# Autodesk Inventor assembly: MQ135
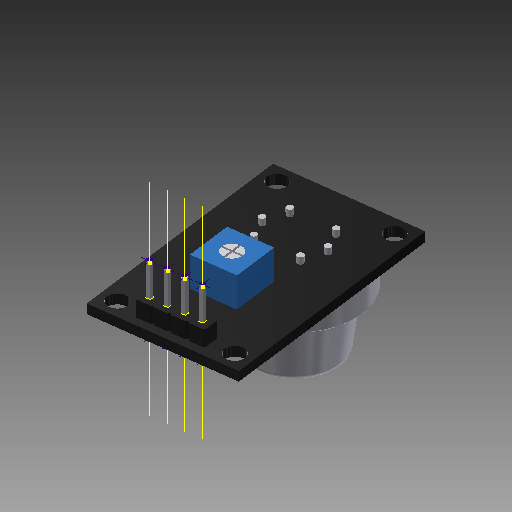
[picture p0: Inventor's stored thumbnail of the model, 512x512]
Saved by Autodesk Inventor 2019 (Build 230136000, 136)
## iProperties
Created: 2019-06-05
Part Number: MQ135
Material: Generisch
Document SubType Name: Assembly
Designer: manue
Author: manue
## Documents named in this file (5)
- E:\Benutzer\manue\Nextcloud\Unterlagen\Studium\OTH AMBERG\Industrie 4.0\Semester 4\Projektmanagement & agile Projektmethoden\Projekt Sensornetzwerk\Sensorknoten\Modell\MQ135\MQ135.iam
- E:\Benutzer\manue\Nextcloud\Unterlagen\Studium\OTH AMBERG\Industrie 4.0\Semester 4\Projektmanagement & agile Projektmethoden\Projekt Sensornetzwerk\Sensorknoten\Modell\MQ135\User Library-MQ135.ipt
- E:\Benutzer\manue\Nextcloud\Unterlagen\Studium\OTH AMBERG\Industrie 4.0\Semester 4\Projektmanagement & agile Projektmethoden\Projekt Sensornetzwerk\Sensorknoten\Modell\MQ135\Platine.ipt
- E:\Benutzer\manue\Nextcloud\Unterlagen\Studium\OTH AMBERG\Industrie 4.0\Semester 4\Projektmanagement & agile Projektmethoden\Projekt Sensornetzwerk\Sensorknoten\Modell\MQ135\Kontaktpins_Gerade.iam
- E:\Benutzer\manue\Nextcloud\Unterlagen\Studium\OTH AMBERG\Industrie 4.0\Semester 4\Projektmanagement & agile Projektmethoden\Projekt Sensornetzwerk\Sensorknoten\Modell\MQ135\Poti.ipt
## Components (7 placed, 4 different names)
1. User Library-MQ135:1 — Passend:4, Passend:5, Zylindrisch:1
2. Platine:1 — Passend:1, Passend:2, Passend:3, Passend:4, Passend:5, Zylindrisch:1, Passend:6, Passend:7, Passend:8
3. Poti:1 — Passend:6, Passend:7, Passend:8
4. Kontaktpins_Gerade:1 [sub-assembly] — Passend:1, Passend:2
5. Kontaktpins_Gerade:2 [sub-assembly]
6. Kontaktpins_Gerade:3 [sub-assembly]
7. Kontaktpins_Gerade:4 [sub-assembly] — Passend:3
## Component patterns: (4 elements, first: Kontaktpins_Gerade:1)
## Relationships (9: Mate 8, CylindricalJoint 1)
- Passend:1 [Mate]: Platine:1 ↔ Kontaktpins_Gerade:1
- Passend:2 [Mate]: Platine:1 ↔ Kontaktpins_Gerade:1
- Passend:3 [Mate]: Platine:1 ↔ Kontaktpins_Gerade:4
- Passend:4 [Mate]: User Library-MQ135:1 ↔ Platine:1
- Passend:5 [Mate]: User Library-MQ135:1 ↔ Platine:1
- Zylindrisch:1 [CylindricalJoint]: User Library-MQ135:1 ↔ Platine:1
- Passend:6 [Mate]: Platine:1 ↔ Poti:1
- Passend:7 [Mate]: Platine:1 ↔ Poti:1
- Passend:8 [Mate]: Platine:1 ↔ Poti:1
